# Autodesk Inventor assembly: [CCW] Gemfan Hurricane 51466
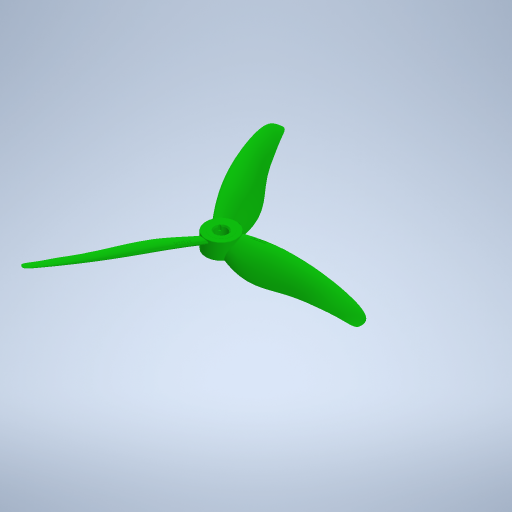
[picture p0: Inventor's stored thumbnail of the model, 512x512]
Saved by Autodesk Inventor 2024 (Build 280153000, 153)
## iProperties
Created: 2024-03-11
Part Number: [CCW] Gemfan Hurricane 51466
Document SubType Name: Assembly
Designer: nicoe
Mass: 3.93079 g
Surface Area: 47.2769 cm^2
Volume: 3.27566 cm^3
Density: 1.2 g/cm^3
Author: nicoe
## Documents named in this file (2)
- D:\users\nicoe\OneDrive\OneDrive - Stellenbosch University\Desktop\Nico_Masters\1. Drone Constrution\CAD Files\Gemfan Hurricane 51466\Gemfan Hurricane 51466\[CCW] Gemfan Hurricane 51466.iam
- D:\users\nicoe\OneDrive\OneDrive - Stellenbosch University\Desktop\Nico_Masters\1. Drone Constrution\CAD Files\Gemfan Hurricane 51466\Gemfan Hurricane 51466\Static (1).ipt
## Components (1 placed, 1 different names)
1. Static (1):1 — Mate:1
## Relationships (3: Mate 2, Angle 1)
- Mate:1: Static (1):1
- Mate:2
- Angle:1 (0 deg)
